# Autodesk Inventor assembly: złożenie pod symulację
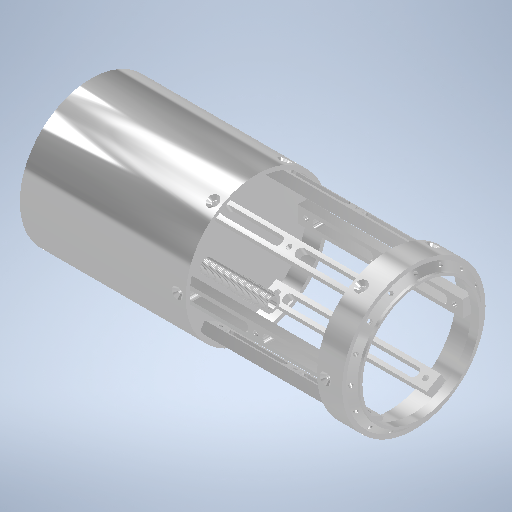
[picture p0: Inventor's stored thumbnail of the model, 512x512]
Saved by Autodesk Inventor 2025.1 (Build 291241020, 241B)
## iProperties
Created: 2024-11-05
Part Number: złożenie pod symulację
Document SubType Name: Assembly
Designer: oem
Author: oem
## Documents named in this file (4)
- C:\Users\oem\Documents\projekty\X simba\złożenie pod symulację.iam
- C:\Users\oem\Documents\projekty\X simba\R7_ENG_2000_OxidizerTank\R7_ENG_2000_OxidizerTank\R7_ENG_2000_OxidizerTank.ipt
- C:\Users\oem\Documents\projekty\X simba\R7_ENG_3101_Bracket\R7_ENG_3101_Bracket\R7_ENG_3101_Bracket.ipt
- C:\Users\oem\Documents\projekty\X simba\Radax prot 3-2\Radax prot 3-2\Radax prot 3-2.ipt
## Components (8 placed, 3 different names)
1. R7_ENG_2000_OxidizerTank:1 — Zestawiające:1, Zestawiające:2
2. Radax prot 3-2:1 — Zestawiające:3, Zestawiające:4
3. R7_ENG_3101_Bracket:1 — Zestawiające:1, Zestawiające:2
4. R7_ENG_3101_Bracket:2
5. R7_ENG_3101_Bracket:3
6. R7_ENG_3101_Bracket:4 — Zestawiające:4
7. R7_ENG_3101_Bracket:5 — Zestawiające:3
8. R7_ENG_3101_Bracket:6
## Component patterns: (6 elements, first: R7_ENG_3101_Bracket:1)
## Relationships (4: Mate 4)
- Zestawiające:1 [Mate]: R7_ENG_2000_OxidizerTank:1 ↔ R7_ENG_3101_Bracket:1
- Zestawiające:2 [Mate]: R7_ENG_2000_OxidizerTank:1 ↔ R7_ENG_3101_Bracket:1
- Zestawiające:3 [Mate]: Radax prot 3-2:1 ↔ R7_ENG_3101_Bracket:5
- Zestawiające:4 [Mate]: Radax prot 3-2:1 ↔ R7_ENG_3101_Bracket:4
